# Autodesk Inventor assembly: VidPad-Case-Only
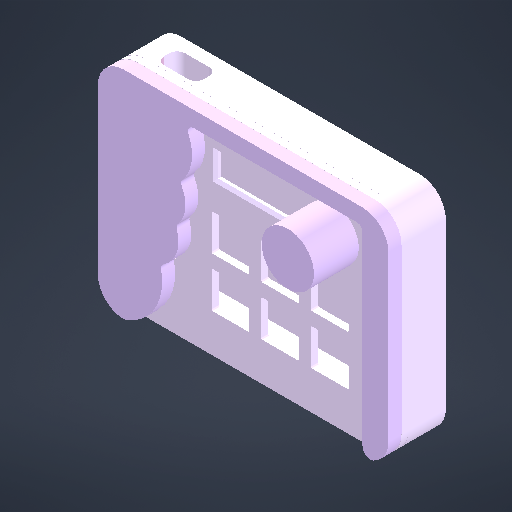
[picture p0: Inventor's stored thumbnail of the model, 512x512]
Saved by Autodesk Inventor 2026.2 (Build 302298000, 298)
## iProperties
Company: Kicad
Created: 2026-02-15
Part Number: VidPad-Case-Only
Description: KiCad electronic assembly
Document SubType Name: Assembly
Designer: bh
Authority: Unknown
Sending System: KiCad to STEP converter
Preprocessor: Open CASCADE STEP processor 7.8
Title: VidPad PCB.step
Author: Pcbnew
## Documents named in this file (5)
- C:\Users\bh\Downloads\VidPad-Case-Only.iam
- C:\Users\bh\Downloads\Top.ipt
- C:\Users\bh\Downloads\RotaryEncoderKnob.ipt
- C:\Users\bh\Downloads\Middle.ipt
- C:\Users\bh\Downloads\Bottom.ipt
## Components (4 placed, 4 different names)
1. Top:1 — Rotational:5
2. RotaryEncoderKnob:1 — Rotational:6
3. Middle:1 — Rotational:4, Rotational:5, Rotational:6
4. Bottom:1 — Rotational:4
## Relationships (3: RevoluteJoint 3)
- Rotational:4 [RevoluteJoint]: Middle:1 ↔ Bottom:1
- Rotational:5 [RevoluteJoint]: Top:1 ↔ Middle:1
- Rotational:6 [RevoluteJoint]: RotaryEncoderKnob:1 ↔ Middle:1
